# Autodesk Inventor assembly: Assy_flame_back
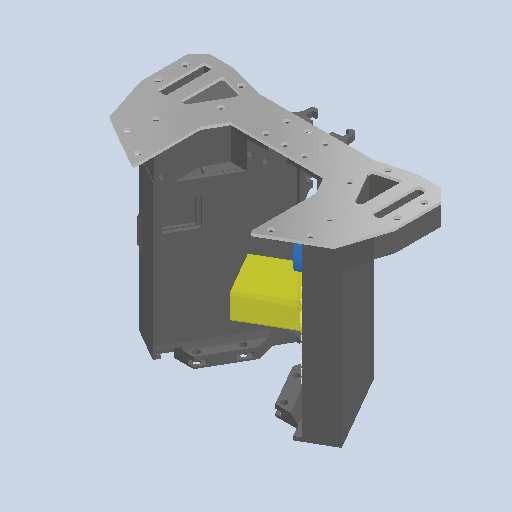
[picture p0: Inventor's stored thumbnail of the model, 512x512]
Saved by Autodesk Inventor 2024.1 (Build 281209000, 209)
## iProperties
Created: 2025-04-23
Part Number: Assy_flame_back
Document SubType Name: Assembly
Designer: hibik
Author: hibik
## Documents named in this file (8)
- C:\Users\hibik\Documents\Robomech\RESCUE\ORCA\hard\flame_back\Assy_flame_back.iam
- C:\Users\hibik\Documents\Robomech\RESCUE\ORCA\hard\flame_back\flame_back.ipt
- C:\Users\hibik\Documents\Robomech\RESCUE\ORCA\hard\flame_back\flame_upper_back.ipt
- C:\Users\hibik\Documents\Robomech\RESCUE\ORCA\hard\flame_back\battery_holder_spring.ipt
- C:\Users\hibik\Documents\Robomech\RESCUE\ORCA\hard\flame_back\battery_holder_cover.ipt
- C:\Users\hibik\Documents\Robomech\RESCUE\ORCA\hard\flame_back\battery_case.ipt
- C:\Users\hibik\Documents\Robomech\RESCUE\ORCA\hard\flame_back\battery_case_cover.ipt
- C:\Users\hibik\Documents\Robomech\RESCUE\ORCA\hard\board\power_model\power.iam
## Components (7 placed, 7 different names)
1. flame_back:1 — 挿入:1, 挿入:2, 挿入:3, 挿入:4, 挿入:5, メイト:1, メイト:2, 角度:1, 挿入:6
2. flame_upper_back:1 — 挿入:1, 挿入:2
3. battery_holder_spring:1 — 挿入:3
4. battery_holder_cover:1 — 挿入:4, 挿入:5
5. battery_case:1 — メイト:1, メイト:2, メイト:3, メイト:4, メイト:5
6. battery_case_cover:1 — メイト:3, メイト:4, メイト:5
7. power:2 [sub-assembly] — 角度:1, 挿入:6
## Relationships (12: Insert 6, Mate 5, Angle 1)
- 挿入:1 [Insert]: flame_back:1 ↔ flame_upper_back:1
- 挿入:2 [Insert]: flame_back:1 ↔ flame_upper_back:1
- 挿入:3 [Insert]: flame_back:1 ↔ battery_holder_spring:1
- 挿入:4 [Insert]: flame_back:1 ↔ battery_holder_cover:1
- 挿入:5 [Insert]: flame_back:1 ↔ battery_holder_cover:1
- メイト:1 [Mate]: flame_back:1 ↔ battery_case:1
- メイト:2 [Mate]: flame_back:1 ↔ battery_case:1
- メイト:3 [Mate]: battery_case:1 ↔ battery_case_cover:1
- メイト:4 [Mate]: battery_case:1 ↔ battery_case_cover:1
- メイト:5 [Mate]: battery_case:1 ↔ battery_case_cover:1
- 角度:1 [Angle] (180 deg): flame_back:1 ↔ power:2
- 挿入:6 [Insert]: flame_back:1 ↔ power:2
